# Autodesk Inventor assembly: Interfas_4
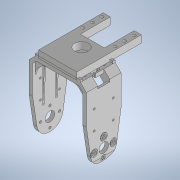
[picture p0: Inventor's stored thumbnail of the model, 180x180]
Saved by Autodesk Inventor 2021.4 (Build 254397000, 397)
## iProperties
Created: 2022-02-03
Part Number: Interfas_4
Document SubType Name: Assembly
Designer: epm01
Author: epm01
## Documents named in this file (3)
- D:\Archivos\2020-2\Papime\Banco_serial\Interfas_4.iam
- D:\Archivos\2020-2\Papime\Banco_serial\FP04-F4.ipt
- D:\Archivos\2020-2\Papime\Banco_serial\Sopoter_gripperM.ipt
## Components (2 placed, 2 different names)
1. FP04-F4:1 — Coincidencia:1, Nivelación:1, Coincidencia:2
2. Sopoter_gripperM:1 — Coincidencia:1, Nivelación:1, Coincidencia:2
## Relationships (3: Mate 2, Flush 1)
- Coincidencia:1 [Mate]: FP04-F4:1 ↔ Sopoter_gripperM:1
- Nivelación:1 [Flush]: FP04-F4:1 ↔ Sopoter_gripperM:1
- Coincidencia:2 [Mate] (3 mm): FP04-F4:1 ↔ Sopoter_gripperM:1
